# Autodesk Inventor assembly: TR2 Arm
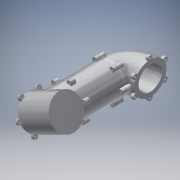
[picture p0: Inventor's stored thumbnail of the model, 180x180]
Saved by Autodesk Inventor 2017 (Build 210142000, 142)
## iProperties
Created: 2018-10-11
Part Number: TR2 Arm
Document SubType Name: Assembly
Designer: Zach
Author: Zach
## Documents named in this file (4)
- C:\Users\Administrator\Documents\GitHub\tr2\Arm\Arm.iam
- C:\Users\Administrator\Documents\GitHub\tr2\Arm\TARM01.ipt
- C:\Users\Administrator\Documents\GitHub\tr2\Arm Actuator\Arm Actuator.iam
- C:\Users\Administrator\Documents\GitHub\tr2\Arm\TARM02.ipt
## Components (3 placed, 3 different names)
1. TARM01:1 — Mate:1, Mate:2, Mate:3
2. Arm Actuator:1 [sub-assembly] — Mate:1, Mate:2, Mate:3, Mate:4, Mate:5, Mate:6
3. TARM02:1 — Mate:4, Mate:5, Mate:6
## Relationships (6: Mate 6)
- Mate:1: TARM01:1 ↔ Arm Actuator:1
- Mate:2: TARM01:1 ↔ Arm Actuator:1
- Mate:3: TARM01:1 ↔ Arm Actuator:1
- Mate:4: Arm Actuator:1 ↔ TARM02:1
- Mate:5: Arm Actuator:1 ↔ TARM02:1
- Mate:6: Arm Actuator:1 ↔ TARM02:1
